# Autodesk Inventor assembly: 装配体
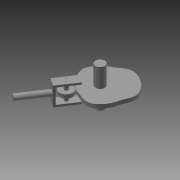
[picture p0: Inventor's stored thumbnail of the model, 180x180]
Saved by Autodesk Inventor 2013 (Build 170138000, 138)
## iProperties
Created: 2012-09-25
Part Number: 装配体
Document SubType Name: Assembly
Designer: Zhensheng
Author: Zhensheng
## Documents named in this file (7)
- E:\inventor\无碳小车\凸轮顶杆转向机构\装配体.iam
- E:\inventor\无碳小车\凸轮顶杆转向机构\凸轮.ipt
- E:\inventor\无碳小车\凸轮顶杆转向机构\滚子.ipt
- E:\inventor\无碳小车\凸轮顶杆转向机构\顶杆.ipt
- E:\inventor\无碳小车\凸轮顶杆转向机构\连接销.ipt
- E:\inventor\无碳小车\凸轮顶杆转向机构\主轴.ipt
- E:\inventor\无碳小车\凸轮顶杆转向机构\套筒.ipt
## Components (6 placed, 6 different names)
1. 凸轮:1 — 表面齐平:1, 插入:2, 角度:1, 角度:2, 角度:3
2. 滚子:1 — 表面齐平:1, 配合:1, 表面齐平:2
3. 顶杆:1 — 插入:1, 配合:2, 表面齐平:2, 角度:2, 角度:3
4. 连接销:1 — 插入:1, 配合:1
5. 主轴:1 — 插入:2
6. 套筒:1 — 配合:2
## Relationships (9: Angle 3, Flush 2, Insert 2, Mate 2)
- 表面齐平:1 [Flush]: 凸轮:1 ↔ 滚子:1
- 插入:1 [Insert]: 顶杆:1 ↔ 连接销:1
- 配合:1 [Mate]: 滚子:1 ↔ 连接销:1
- 插入:2 [Insert] (-10 mm): 凸轮:1 ↔ 主轴:1
- 配合:2 [Mate]: 顶杆:1 ↔ 套筒:1
- 角度:1 [Angle] (90 deg): 凸轮:1
- 表面齐平:2 [Flush] (4 mm): 滚子:1 ↔ 顶杆:1
- 角度:2 [Angle] (90 deg): 凸轮:1 ↔ 顶杆:1
- 角度:3 [Angle] (90 deg): 凸轮:1 ↔ 顶杆:1
